# Autodesk Inventor assembly: Assembly1
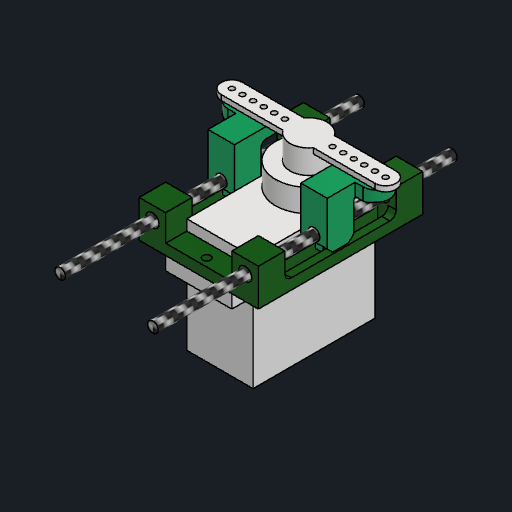
[picture p0: Inventor's stored thumbnail of the model, 512x512]
Saved by Autodesk Inventor 2023 (Build 270158000, 158)
## iProperties
Created: 2022-07-10
Part Number: Assembly1
Document SubType Name: Assembly
Designer: legot
Author: legot
## Documents named in this file (7)
- C:\Users\legot\Documents\Inventor\HIKOSAPO\Drop\om_Drop_10g.iam
- C:\Users\legot\Documents\Inventor\HIKOSAPO\public_parts\ServoMotor_10g.ipt
- C:\Users\legot\Documents\Inventor\HIKOSAPO\Drop\om_DropBase_10g.ipt
- C:\Users\legot\Documents\Inventor\HIKOSAPO\public_parts\horn_10g.ipt
- C:\Users\legot\Documents\Inventor\HIKOSAPO\Drop\om_Drop_10g_L.ipt
- C:\Users\legot\Documents\Inventor\HIKOSAPO\Drop\om_Drop_10g_R.ipt
- C:\Users\legot\Documents\Inventor\HIKOSAPO\Drop\om_Drop_shaft_10g.ipt
## Components (7 placed, 6 different names)
1. ServoMotor_10g:1 — メイト:1, メイト:2, 挿入:1, メイト:8
2. om_DropBase_10g:1 — メイト:1, メイト:2, メイト:4, フラッシュ:1, メイト:5, フラッシュ:2, メイト:8, 角度:1
3. horn_10g:1 — 挿入:1, メイト:9, メイト:10, 角度:1
4. om_Drop_10g_L:1 — メイト:4, フラッシュ:1, メイト:9, 挿入:2
5. om_Drop_10g_R:1 — メイト:5, フラッシュ:2, メイト:10, 挿入:3
6. om_Drop_shaft_10g:1 — 挿入:2
7. om_Drop_shaft_10g:2 — 挿入:3
## Relationships (13: Mate 7, Insert 3, Flush 2, Angle 1)
- メイト:1 [Mate]: ServoMotor_10g:1 ↔ om_DropBase_10g:1
- メイト:2 [Mate]: ServoMotor_10g:1 ↔ om_DropBase_10g:1
- 挿入:1 [Insert]: ServoMotor_10g:1 ↔ horn_10g:1
- メイト:4 [Mate]: om_DropBase_10g:1 ↔ om_Drop_10g_L:1
- フラッシュ:1 [Flush]: om_DropBase_10g:1 ↔ om_Drop_10g_L:1
- メイト:5 [Mate]: om_DropBase_10g:1 ↔ om_Drop_10g_R:1
- フラッシュ:2 [Flush]: om_DropBase_10g:1 ↔ om_Drop_10g_R:1
- メイト:8 [Mate]: ServoMotor_10g:1 ↔ om_DropBase_10g:1
- メイト:9 [Mate]: horn_10g:1 ↔ om_Drop_10g_L:1
- メイト:10 [Mate]: horn_10g:1 ↔ om_Drop_10g_R:1
- 挿入:2 [Insert] (-21 mm): om_Drop_10g_L:1 ↔ om_Drop_shaft_10g:1
- 挿入:3 [Insert] (-21 mm): om_Drop_10g_R:1 ↔ om_Drop_shaft_10g:2
- 角度:1 [Angle] (0 deg): om_DropBase_10g:1 ↔ horn_10g:1
